# Autodesk Inventor assembly: assembly_hand
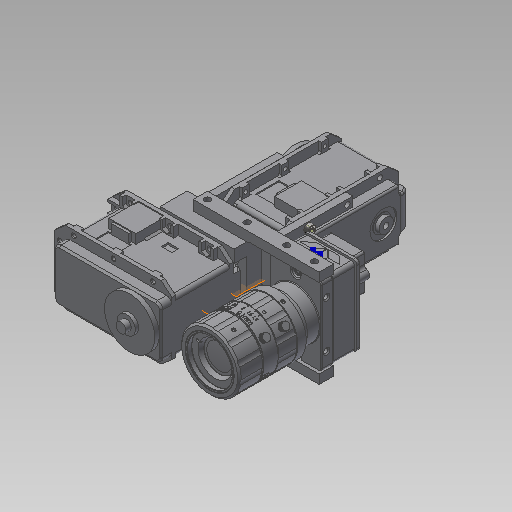
[picture p0: Inventor's stored thumbnail of the model, 512x512]
Saved by Autodesk Inventor 2017 (Build 210142000, 142)
## iProperties
Part Number: assembly_hand
Material: Generisch
Document SubType Name: Assembly
Designer: Max
Author: Max
## Documents named in this file (7)
- C:\Users\Max\Desktop\SENAI\robot_arm_new\assembly_hand.iam
- C:\Users\Max\Desktop\SENAI\robot_arm_new\MX-106T.ipt
- C:\Users\Max\Desktop\SENAI\robot_arm_new\connection_hand.ipt
- C:\Users\Max\Desktop\SENAI\robot_arm_new\connection_hand_2.ipt
- C:\Users\Max\Desktop\SENAI\robot_arm_new\assembly_camera.iam
- C:\Users\Max\Documents\Inventor\Content Center Files\R2017\de-DE\DIN 912\DIN 912 - M2,5 x 0,45 x 6 x 4,875.ipt
- C:\Users\Max\Desktop\SENAI\robot_arm_new\connection_hand_camera.ipt
## Components (9 placed, 6 different names)
1. MX-106T:1 — Passend:1, Passend:2, Passend:3, Passend:10, Passend:11
2. MX-106T:2 — Passend:7, Passend:8, Passend:9
3. connection_hand:1 — Passend:1, Passend:2, Passend:3, Passend:4, Passend:5, Passend:6, Passend:14, Passend:15, Passend:16, Passend:17
4. connection_hand_2:1 — Passend:4, Passend:5, Passend:6, Passend:7, Passend:8, Passend:9, Passend:18, Passend:19, Passend:20, Passend:26, Passend:27, Passend:29
5. assembly_camera:1 [sub-assembly] — Passend:21, Passend:22, Passend:23, Passend:24, Passend:25, Passend:28
6. DIN 912 - ersetzt durch DIN EN ISO 4762 M2,5 x 6:1 — Passend:15, Passend:17
7. DIN 912 - ersetzt durch DIN EN ISO 4762 M2,5 x 6:3 — Passend:14, Passend:16
8. connection_hand_camera:1 — Passend:18, Passend:19, Passend:20, Passend:21, Passend:22, Passend:23
9. connection_hand_camera:2 — Passend:24, Passend:25, Passend:26, Passend:27, Passend:28, Passend:29
## Relationships (27: Mate 27)
- Passend:1 [Mate]: MX-106T:1 ↔ connection_hand:1
- Passend:2 [Mate]: MX-106T:1 ↔ connection_hand:1
- Passend:3 [Mate]: MX-106T:1 ↔ connection_hand:1
- Passend:4 [Mate]: connection_hand:1 ↔ connection_hand_2:1
- Passend:5 [Mate]: connection_hand:1 ↔ connection_hand_2:1
- Passend:6 [Mate]: connection_hand:1 ↔ connection_hand_2:1
- Passend:7 [Mate]: MX-106T:2 ↔ connection_hand_2:1
- Passend:8 [Mate]: MX-106T:2 ↔ connection_hand_2:1
- Passend:9 [Mate]: MX-106T:2 ↔ connection_hand_2:1
- Passend:10 [Mate]: MX-106T:1
- Passend:11 [Mate]: MX-106T:1
- Passend:14 [Mate]: connection_hand:1 ↔ DIN 912 - ersetzt durch DIN EN ISO 4762 M2,5 x 6:3
- Passend:15 [Mate]: connection_hand:1 ↔ DIN 912 - ersetzt durch DIN EN ISO 4762 M2,5 x 6:1
- Passend:16 [Mate]: connection_hand:1 ↔ DIN 912 - ersetzt durch DIN EN ISO 4762 M2,5 x 6:3
- Passend:17 [Mate]: connection_hand:1 ↔ DIN 912 - ersetzt durch DIN EN ISO 4762 M2,5 x 6:1
- Passend:18 [Mate]: connection_hand_2:1 ↔ connection_hand_camera:1
- Passend:19 [Mate]: connection_hand_2:1 ↔ connection_hand_camera:1
- Passend:20 [Mate]: connection_hand_2:1 ↔ connection_hand_camera:1
- Passend:21 [Mate]: assembly_camera:1 ↔ connection_hand_camera:1
- Passend:22 [Mate]: assembly_camera:1 ↔ connection_hand_camera:1
- Passend:23 [Mate]: assembly_camera:1 ↔ connection_hand_camera:1
- Passend:24 [Mate]: assembly_camera:1 ↔ connection_hand_camera:2
- Passend:25 [Mate]: assembly_camera:1 ↔ connection_hand_camera:2
- Passend:26 [Mate]: connection_hand_2:1 ↔ connection_hand_camera:2
- Passend:27 [Mate]: connection_hand_2:1 ↔ connection_hand_camera:2
- Passend:28 [Mate]: assembly_camera:1 ↔ connection_hand_camera:2
- Passend:29 [Mate]: connection_hand_2:1 ↔ connection_hand_camera:2
